# Autodesk Inventor assembly: Assembly.
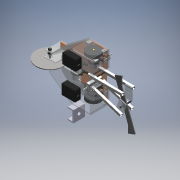
[picture p0: Inventor's stored thumbnail of the model, 180x180]
Saved by Autodesk Inventor 2019 (Build 230136000, 136)
## iProperties
Created: 2018-08-16
Part Number: Assembly.
Document SubType Name: Assembly
Designer: andres2416
Author: andres2416
## Documents named in this file (26)
- C:\Users\garstka1245\Downloads\robot\full-bot-assembly.iam
- C:\Users\garstka1245\Downloads\robot\Electronics\battery.ipt
- C:\Users\garstka1245\Downloads\robot\Motor Mount H\motor-mount-h-E30-bot.ipt
- C:\Users\garstka1245\Downloads\robot\Motor Mount H\motor-mount-h-E30-top.ipt
- C:\Users\garstka1245\Downloads\robot\Mechanicals\motor-E30-400.ipt
- C:\Users\garstka1245\Downloads\robot\Structure\bar-aluminium.ipt
- C:\Users\garstka1245\Downloads\robot\Structure\standoff.ipt
- C:\Users\garstka1245\Downloads\robot\Weapon Saw\wall-side-saw.ipt
- C:\Users\garstka1245\Downloads\robot\Weapon Saw\wall-saw-support.ipt
- C:\Users\garstka1245\Downloads\robot\Weapon Saw\wall-side-saw-hole.ipt
- C:\Users\garstka1245\Downloads\robot\Weapon Saw\weapon-saw.ipt
- C:\Users\garstka1245\Downloads\robot\Mechanicals\wheel-6in.ipt
- C:\Users\garstka1245\Downloads\robot\Weapon Saw\axle-saw.ipt
- C:\Users\garstka1245\Downloads\robot\Shell\base\base.ipt
- C:\Users\garstka1245\Downloads\robot\Shell\second-layer\platform.ipt
- C:\Users\garstka1245\Downloads\robot\Mechanicals\gear-vex.ipt
- C:\Users\garstka1245\Downloads\robot\Weapon Saw\axle-shaft-collar-saw.ipt
- C:\Users\garstka1245\Downloads\robot\Weapon Spinner\mount-point.ipt
- C:\Users\garstka1245\Downloads\robot\Weapon Spinner\axle-spinner.ipt
- C:\Users\garstka1245\Downloads\robot\Weapon Spinner\weapon-spinner.ipt
- C:\Users\garstka1245\Downloads\robot\Shell\wall-parts\wall-spinner.ipt
- C:\Users\garstka1245\Downloads\robot\Shell\wall-parts\wall-side.ipt
- C:\Users\garstka1245\Downloads\robot\Shell\wall-parts\wall-angled.ipt
- C:\Users\garstka1245\Downloads\robot\Structure\bracket-aluminium.ipt
- C:\Users\garstka1245\Downloads\robot\Motor Mount V\motor-mount-v-E30.ipt
- C:\Users\garstka1245\Downloads\robot\Mechanicals\pillowblock.ipt
## Components (61 placed, 25 different names)
1. battery:1
2. battery:3 — Mate:11, Flush:22
3. wheel-6in:2 — Rotation:3
4. wheel-6in:1 — Insert:42, Rotation:3
5. gear-vex:1 — Insert:47
6. gear-vex:2 — Insert:55
7. pillowblock:1
8. pillowblock:2
9. motor-E30-400:1 — Insert:8, Insert:42, Insert:51
10. motor-E30-400:2
11. motor-E30-400:3 — Insert:48, Tangent:50, Insert:50, Insert:55
12. motor-mount-h-E30-bot:1 — Insert:8, Flush:15
13. motor-mount-h-E30-bot:2
14. motor-mount-h-E30-top:2 — Insert:11, Insert:12
15. motor-mount-h-E30-bot:3 — Insert:11, Insert:12
16. motor-mount-h-E30-top:3 — Insert:13, Insert:14
17. motor-mount-h-E30-bot:4 — Insert:13, Insert:14
18. motor-mount-h-E30-bot:5 — Mate:6, Flush:11, Flush:12, Mate:8, Flush:14
19. motor-mount-h-E30-top:7 — Mate:8, Insert:50, Flush:14
20. motor-mount-h-E30-bot:6 — Mate:5, Flush:9, Flush:10, Flush:12, Insert:48, Mate:7, Flush:13
21. motor-mount-h-E30-top:8 — Mate:7, Tangent:50, Flush:13
22. motor-mount-h-E30-top:5 — Insert:51, Flush:15, Insert:52, Mate:9, Flush:18
23. motor-mount-h-E30-top:6 — Insert:52, Flush:19
24. motor-mount-v-E30:1 — Insert:66, Insert:67
25. platform:2 — Mate:9, Flush:18, Flush:19, Mate:11, Flush:22
26. platform:1
27. base:1 — Insert:33, Insert:36, Mate:3, Flush:6, Mate:4, Flush:7, Flush:8, Mate:5, Flush:9, Flush:10, Mate:6, Flush:11, Mate:14, Flush:27, Flush:28, Mate:16, Flush:31, Mate:20, Flush:33, Mate:22, Flush:34, Insert:56, Insert:57, Insert:58, Insert:59, Mate:28, Flush:36, Insert:60, Insert:61, Insert:62, Insert:63, Mate:33, Flush:37, Insert:64, Insert:65, Insert:66, Insert:67
28. wall-side:1 — Mate:16, Flush:31, Mate:21, Flush:35, Mate:31, Mate:32
29. wall-side:2 — Mate:33, Mate:34, Flush:37, Mate:35, Mate:36
30. wall-spinner:1 — Mate:28, Flush:35, Flush:36, Mate:29, Mate:30, Mate:34
31. wall-angled:2 — Mate:20, Flush:33, Mate:21, Mate:25, Mate:26
32. wall-angled:1 — Mate:22, Flush:34, Mate:24, Mate:27
33. standoff:4 — Insert:24, Insert:26
34. standoff:3 — Insert:23, Insert:25
35. standoff:2 — Insert:22, Insert:28
36. standoff:1 — Insert:21, Insert:27
37. bar-aluminium:1 — Insert:23, Insert:24, Insert:36
38. bar-aluminium:2 — Insert:21, Insert:22, Insert:33, Mate:12, Flush:23, Flush:24
39. bar-aluminium:3 — Insert:25, Insert:26, Flush:25, Flush:26
40. bar-aluminium:4 — Insert:27, Insert:28, Mate:13
41. bracket-aluminium:1 — Insert:56, Mate:24
42. bracket-aluminium:2 — Insert:57, Mate:27
43. bracket-aluminium:3 — Insert:58, Mate:25
44. bracket-aluminium:4 — Insert:59, Mate:26
45. bracket-aluminium:5 — Insert:61, Mate:30
46. bracket-aluminium:6 — Insert:60, Mate:29
47. bracket-aluminium:7 — Insert:65, Mate:36
48. bracket-aluminium:8 — Insert:64, Mate:35
49. bracket-aluminium:9 — Insert:63, Mate:32
50. bracket-aluminium:10 — Insert:62, Mate:31
51. wall-side-saw-hole:1 — Mate:4, Flush:7, Flush:8, Insert:45, Insert:46
52. wall-saw-support:1 — Mate:3, Flush:6, Insert:43
53. wall-side-saw:1 — Mate:14, Flush:27, Flush:28
54. weapon-saw:1 — Insert:43, Insert:44
55. axle-saw:1 — Insert:44, Insert:47
56. axle-shaft-collar-saw:1 — Insert:45
57. axle-shaft-collar-saw:2 — Insert:46
58. mount-point:1 — Mate:13, Flush:25, Flush:26, Insert:53
59. mount-point:2 — Mate:12, Flush:23, Flush:24
60. axle-spinner:1 — Insert:53, Rotation:2, Insert:54
61. weapon-spinner:1 — Rotation:2, Insert:54
## Relationships (96: Insert 40, Mate 28, Flush 25, RelateRotation 2, Tangent 1)
- Insert:8 (-12.7 mm): motor-E30-400:1 ↔ motor-mount-h-E30-bot:1
- Insert:11: motor-mount-h-E30-top:2 ↔ motor-mount-h-E30-bot:3
- Insert:12: motor-mount-h-E30-top:2 ↔ motor-mount-h-E30-bot:3
- Insert:13: motor-mount-h-E30-top:3 ↔ motor-mount-h-E30-bot:4
- Insert:14: motor-mount-h-E30-top:3 ↔ motor-mount-h-E30-bot:4
- Insert:21: standoff:1 ↔ bar-aluminium:2
- Insert:22: standoff:2 ↔ bar-aluminium:2
- Insert:23: standoff:3 ↔ bar-aluminium:1
- Insert:24: standoff:4 ↔ bar-aluminium:1
- Insert:25: standoff:3 ↔ bar-aluminium:3
- Insert:26: standoff:4 ↔ bar-aluminium:3
- Insert:27: standoff:1 ↔ bar-aluminium:4
- Insert:28: standoff:2 ↔ bar-aluminium:4
- Insert:33: base:1 ↔ bar-aluminium:2
- Insert:36: base:1 ↔ bar-aluminium:1
- Insert:42 (-38.1 mm): wheel-6in:1 ↔ motor-E30-400:1
- Mate:3: base:1 ↔ wall-saw-support:1
- Flush:6: base:1 ↔ wall-saw-support:1
- Mate:4: base:1 ↔ wall-side-saw-hole:1
- Flush:7: base:1 ↔ wall-side-saw-hole:1
- Flush:8: base:1 ↔ wall-side-saw-hole:1
- Insert:43 (7.62 mm): wall-saw-support:1 ↔ weapon-saw:1
- Insert:44 (-114.3 mm): weapon-saw:1 ↔ axle-saw:1
- Insert:45: wall-side-saw-hole:1 ↔ axle-shaft-collar-saw:1
- Insert:46: wall-side-saw-hole:1 ↔ axle-shaft-collar-saw:2
- Insert:47 (-101.6 mm): gear-vex:1 ↔ axle-saw:1
- Mate:5: motor-mount-h-E30-bot:6 ↔ base:1
- Flush:9 (177.8 mm): motor-mount-h-E30-bot:6 ↔ base:1
- Flush:10 (165.1 mm): motor-mount-h-E30-bot:6 ↔ base:1
- Mate:6: motor-mount-h-E30-bot:5 ↔ base:1
- Flush:11 (-241.3 mm): motor-mount-h-E30-bot:5 ↔ base:1
- Flush:12: motor-mount-h-E30-bot:5 ↔ motor-mount-h-E30-bot:6
- Insert:48 (-63.5 mm): motor-E30-400:3 ↔ motor-mount-h-E30-bot:6
- Mate:7: motor-mount-h-E30-bot:6 ↔ motor-mount-h-E30-top:8
- Tangent:50: motor-E30-400:3 ↔ motor-mount-h-E30-top:8
- Flush:13: motor-mount-h-E30-bot:6 ↔ motor-mount-h-E30-top:8
- Mate:8: motor-mount-h-E30-bot:5 ↔ motor-mount-h-E30-top:7
- Insert:50: motor-E30-400:3 ↔ motor-mount-h-E30-top:7
- Flush:14: motor-mount-h-E30-bot:5 ↔ motor-mount-h-E30-top:7
- Insert:51: motor-E30-400:1 ↔ motor-mount-h-E30-top:5
- Flush:15: motor-mount-h-E30-bot:1 ↔ motor-mount-h-E30-top:5
- Insert:52 (38.1 mm): motor-mount-h-E30-top:5 ↔ motor-mount-h-E30-top:6
- Mate:9: motor-mount-h-E30-top:5 ↔ platform:2
- Flush:18: motor-mount-h-E30-top:5 ↔ platform:2
- Flush:19 (-29.21 mm): motor-mount-h-E30-top:6 ↔ platform:2
- Mate:11: battery:3 ↔ platform:2
- Flush:22 (25.4 mm): battery:3 ↔ platform:2
- Mate:12: bar-aluminium:2 ↔ mount-point:2
- Flush:23: bar-aluminium:2 ↔ mount-point:2
- Flush:24: bar-aluminium:2 ↔ mount-point:2
- Mate:13: bar-aluminium:4 ↔ mount-point:1
- Flush:25: bar-aluminium:3 ↔ mount-point:1
- Flush:26: bar-aluminium:3 ↔ mount-point:1
- Insert:53 (-19.05 mm): mount-point:1 ↔ axle-spinner:1
- Rotation:2 [RelateRotation] (1 ul): axle-spinner:1 ↔ weapon-spinner:1
- Insert:54 (50.8 mm): axle-spinner:1 ↔ weapon-spinner:1
- Rotation:3 [RelateRotation] (1 ul): wheel-6in:2 ↔ wheel-6in:1
- Mate:14: base:1 ↔ wall-side-saw:1
- Flush:27: base:1 ↔ wall-side-saw:1
- Flush:28: base:1 ↔ wall-side-saw:1
- Insert:55 (-34.29 mm): gear-vex:2 ↔ motor-E30-400:3
- Mate:16: base:1 ↔ wall-side:1
- Flush:31: base:1 ↔ wall-side:1
- Mate:20: base:1 ↔ wall-angled:2
- Flush:33: base:1 ↔ wall-angled:2
- Mate:21: wall-side:1 ↔ wall-angled:2
- Mate:22: base:1 ↔ wall-angled:1
- Flush:34: base:1 ↔ wall-angled:1
- Insert:56: base:1 ↔ bracket-aluminium:1
- Mate:24: wall-angled:1 ↔ bracket-aluminium:1
- Insert:57: base:1 ↔ bracket-aluminium:2
- Insert:58: base:1 ↔ bracket-aluminium:3
- Insert:59: base:1 ↔ bracket-aluminium:4
- Mate:25: wall-angled:2 ↔ bracket-aluminium:3
- Mate:26: wall-angled:2 ↔ bracket-aluminium:4
- Mate:27: wall-angled:1 ↔ bracket-aluminium:2
- Mate:28: base:1 ↔ wall-spinner:1
- Flush:35: wall-side:1 ↔ wall-spinner:1
- Flush:36: base:1 ↔ wall-spinner:1
- Insert:60: base:1 ↔ bracket-aluminium:6
- Mate:29: wall-spinner:1 ↔ bracket-aluminium:6
- Insert:61: base:1 ↔ bracket-aluminium:5
- Mate:30: wall-spinner:1 ↔ bracket-aluminium:5
- Insert:62: base:1 ↔ bracket-aluminium:10
- Mate:31: wall-side:1 ↔ bracket-aluminium:10
- Insert:63: base:1 ↔ bracket-aluminium:9
- Mate:32: wall-side:1 ↔ bracket-aluminium:9
- Mate:33: base:1 ↔ wall-side:2
- Mate:34: wall-side:2 ↔ wall-spinner:1
- Flush:37: base:1 ↔ wall-side:2
- Insert:64: base:1 ↔ bracket-aluminium:8
- Mate:35: wall-side:2 ↔ bracket-aluminium:8
- Insert:65: base:1 ↔ bracket-aluminium:7
- Mate:36: wall-side:2 ↔ bracket-aluminium:7
- Insert:66: motor-mount-v-E30:1 ↔ base:1
- Insert:67: motor-mount-v-E30:1 ↔ base:1
